# Autodesk Inventor assembly: omni-rover-rev2
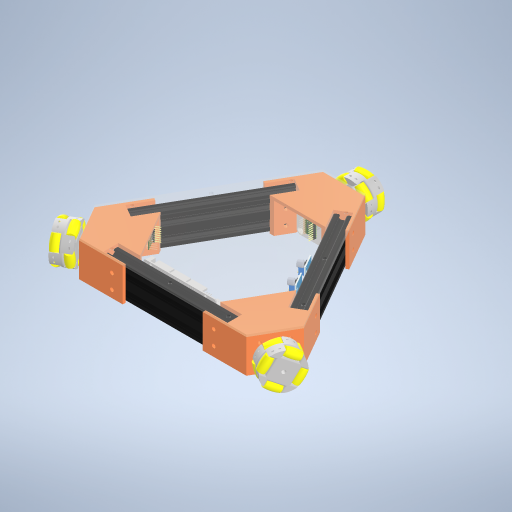
[picture p0: Inventor's stored thumbnail of the model, 512x512]
Saved by Autodesk Inventor 2024.2 (Build 282272000, 272)
## iProperties
Created: 2024-03-31
Part Number: omni-rover-rev2
Document SubType Name: Assembly
Designer: Robin
Mass: 1494.17 g
Surface Area: 6342.82 cm^2
Volume: 1204.42 cm^3
Density: 1.24057 g/cm^3
Author: Robin
## Documents named in this file (9)
- C:\Users\Robin\Documents\MechanicalDesign\CAD\omni-rover-rev2.iam
- C:\Users\Robin\Documents\MechanicalDesign\CAD\cornerBracket.ipt
- C:\Users\Robin\Documents\MechanicalDesign\CAD\2040aluminum_extrusion_black.ipt
- C:\Users\Robin\Documents\MechanicalDesign\CAD\acrylic.ipt
- C:\Users\Robin\Documents\MechanicalDesign\CAD\Nema-17\NEMA17\Inventor\17HM15-0904S.iam
- C:\Users\Robin\Documents\MechanicalDesign\CAD\ArduinoMega_STEP_AP203\ArduinoMega_STEP_AP203.ipt
- C:\Users\Robin\Documents\MechanicalDesign\CAD\tmc2209-stepper-motor-driver-1\TMC2209 V3.0\TMC2209 V3.0.ipt
- C:\Users\Robin\Documents\MechanicalDesign\CAD\buck-converter-7\LM2596 DC to DC Buck Converter 3 A\LM2596 DC to DC Buck Converter 3 A.ipt
- C:\Users\Robin\Documents\MechanicalDesign\CAD\omni-wheel-90deg.iam
## Components (19 placed, 8 different names)
1. cornerBracket:1 — Mate:17, Mate:18, Mate:19, Mate:20, Mate:21, Mate:25, Mate:26, Angle:1, Mate:35, Mate:44, Mate:45, Mate:53
2. cornerBracket:2 — Mate:5, Mate:6, Mate:7, Mate:8, Mate:11, Mate:12, Mate:22, Mate:23, Angle:3, Mate:42, Mate:43, Mate:48, Mate:55
3. cornerBracket:3 — Mate:9, Mate:10, Mate:13, Mate:14, Mate:15, Mate:16, Flush:1, Flush:2, Mate:24, Angle:2, Mate:29, Mate:46, Mate:47, Mate:54
4. 2040aluminum_extrusion_black:1 — Mate:5, Mate:6, Mate:12, Mate:21, Mate:34
5. 2040aluminum_extrusion_black:2 — Mate:14, Mate:15, Mate:16, Mate:17, Mate:18, Mate:19
6. 2040aluminum_extrusion_black:3 — Mate:7, Mate:8, Mate:9, Mate:10, Mate:11, Mate:13, Mate:40, Mate:41, Flush:5
7. acrylic:1 — Flush:1, Mate:20, Flush:2, Flush:3, Mate:36
8. 17HM15-0904S:1 [sub-assembly] — Mate:24, Angle:2, Mate:29, Mate:39, Mate:51
9. 17HM15-0904S:2 [sub-assembly] — Mate:25, Mate:26, Angle:1, Mate:38, Mate:52
10. 17HM15-0904S:3 [sub-assembly] — Mate:22, Mate:23, Angle:3, Mate:37, Mate:50
11. ArduinoMega_STEP_AP203:1 — Mate:34, Mate:35, Mate:36
12. TMC2209 V3.0:1 — Mate:38, Mate:44, Mate:45
13. TMC2209 V3.0:2 — Mate:37, Mate:42, Mate:43
14. TMC2209 V3.0:3 — Mate:39, Mate:46, Mate:47
15. LM2596 DC to DC Buck Converter 3 A:1 — Mate:40, Mate:48, Mate:49, Flush:4
16. LM2596 DC to DC Buck Converter 3 A:2 — Mate:41, Mate:49, Flush:4, Flush:5
17. omni-wheel-90deg:1 [sub-assembly] — Mate:50, Mate:55
18. omni-wheel-90deg:2 [sub-assembly] — Mate:52, Mate:53
19. omni-wheel-90deg:3 [sub-assembly] — Mate:51, Mate:54
## Relationships (53: Mate 45, Flush 5, Angle 3)
- Mate:5: cornerBracket:2 ↔ 2040aluminum_extrusion_black:1
- Mate:6: cornerBracket:2 ↔ 2040aluminum_extrusion_black:1
- Mate:7: cornerBracket:2 ↔ 2040aluminum_extrusion_black:3
- Mate:8: cornerBracket:2 ↔ 2040aluminum_extrusion_black:3
- Mate:9: cornerBracket:3 ↔ 2040aluminum_extrusion_black:3
- Mate:10: cornerBracket:3 ↔ 2040aluminum_extrusion_black:3
- Mate:11: cornerBracket:2 ↔ 2040aluminum_extrusion_black:3
- Mate:12: cornerBracket:2 ↔ 2040aluminum_extrusion_black:1
- Mate:13: cornerBracket:3 ↔ 2040aluminum_extrusion_black:3
- Mate:14: cornerBracket:3 ↔ 2040aluminum_extrusion_black:2
- Mate:15: cornerBracket:3 ↔ 2040aluminum_extrusion_black:2
- Mate:16: cornerBracket:3 ↔ 2040aluminum_extrusion_black:2
- Mate:17: cornerBracket:1 ↔ 2040aluminum_extrusion_black:2
- Mate:18: cornerBracket:1 ↔ 2040aluminum_extrusion_black:2
- Mate:19: cornerBracket:1 ↔ 2040aluminum_extrusion_black:2
- Flush:1: cornerBracket:3 ↔ acrylic:1
- Mate:20: cornerBracket:1 ↔ acrylic:1
- Mate:21: cornerBracket:1 ↔ 2040aluminum_extrusion_black:1
- Flush:2: cornerBracket:3 ↔ acrylic:1
- Mate:22: cornerBracket:2 ↔ 17HM15-0904S:3
- Mate:23: cornerBracket:2 ↔ 17HM15-0904S:3
- Mate:24: cornerBracket:3 ↔ 17HM15-0904S:1
- Mate:25: cornerBracket:1 ↔ 17HM15-0904S:2
- Mate:26: cornerBracket:1 ↔ 17HM15-0904S:2
- Angle:1 (0 deg): cornerBracket:1 ↔ 17HM15-0904S:2
- Angle:2 (0 deg): cornerBracket:3 ↔ 17HM15-0904S:1
- Angle:3 (0 deg): cornerBracket:2 ↔ 17HM15-0904S:3
- Mate:29: cornerBracket:3 ↔ 17HM15-0904S:1
- Flush:3: acrylic:1
- Mate:34: 2040aluminum_extrusion_black:1 ↔ ArduinoMega_STEP_AP203:1
- Mate:35 (32 mm): cornerBracket:1 ↔ ArduinoMega_STEP_AP203:1
- Mate:36 (1 mm): acrylic:1 ↔ ArduinoMega_STEP_AP203:1
- Mate:37 (15 mm): 17HM15-0904S:3 ↔ TMC2209 V3.0:2
- Mate:38 (15 mm): 17HM15-0904S:2 ↔ TMC2209 V3.0:1
- Mate:39 (15 mm): 17HM15-0904S:1 ↔ TMC2209 V3.0:3
- Mate:40 (1 mm): 2040aluminum_extrusion_black:3 ↔ LM2596 DC to DC Buck Converter 3 A:1
- Mate:41: 2040aluminum_extrusion_black:3 ↔ LM2596 DC to DC Buck Converter 3 A:2
- Mate:42 (2 mm): cornerBracket:2 ↔ TMC2209 V3.0:2
- Mate:43 (2 mm): cornerBracket:2 ↔ TMC2209 V3.0:2
- Mate:44: cornerBracket:1 ↔ TMC2209 V3.0:1
- Mate:45: cornerBracket:1 ↔ TMC2209 V3.0:1
- Mate:46: cornerBracket:3 ↔ TMC2209 V3.0:3
- Mate:47: cornerBracket:3 ↔ TMC2209 V3.0:3
- Mate:48 (35 mm): cornerBracket:2 ↔ LM2596 DC to DC Buck Converter 3 A:1
- Mate:49 (10 mm): LM2596 DC to DC Buck Converter 3 A:1 ↔ LM2596 DC to DC Buck Converter 3 A:2
- Flush:4: LM2596 DC to DC Buck Converter 3 A:1 ↔ LM2596 DC to DC Buck Converter 3 A:2
- Flush:5 (-3 mm): 2040aluminum_extrusion_black:3 ↔ LM2596 DC to DC Buck Converter 3 A:2
- Mate:50: 17HM15-0904S:3 ↔ omni-wheel-90deg:1
- Mate:51: 17HM15-0904S:1 ↔ omni-wheel-90deg:3
- Mate:52: 17HM15-0904S:2 ↔ omni-wheel-90deg:2
- Mate:53 (2 mm): cornerBracket:1 ↔ omni-wheel-90deg:2
- Mate:54 (2 mm): cornerBracket:3 ↔ omni-wheel-90deg:3
- Mate:55 (2 mm): cornerBracket:2 ↔ omni-wheel-90deg:1
